# Autodesk Inventor assembly: AluminumProfileMount
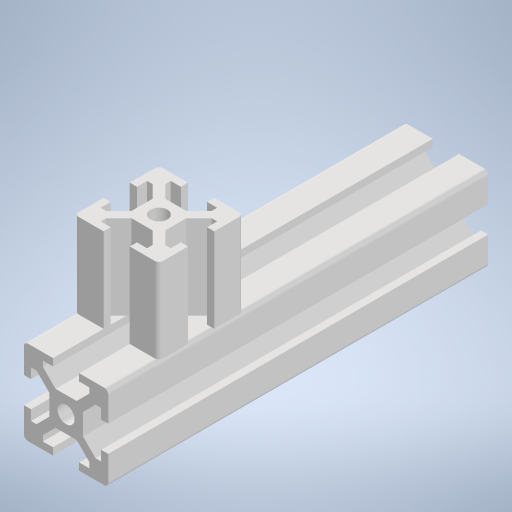
[picture p0: Inventor's stored thumbnail of the model, 512x512]
Saved by Autodesk Inventor 2023 (Build 270158000, 158)
## iProperties
Created: 2024-02-04
Part Number: AluminumProfileMount
Document SubType Name: Assembly
Designer: victo
Author: victo
## Documents named in this file (3)
- C:\Users\victo\Documents\ball-balancing-digital-twin\Mechanics\CAD\AluminumProfileMount.iam
- C:\Users\victo\Documents\ball-balancing-digital-twin\Mechanics\CAD\Aluminum_Profile_202090.ipt
- C:\Users\victo\Documents\ball-balancing-digital-twin\Mechanics\CAD\Aluminum_Profile_202020.ipt
## Components (2 placed, 2 different names)
1. Aluminum_Profile_202090:1 — Mate:1, Flush:1, Flush:2
2. Aluminum_Profile_202020:1 — Mate:1, Flush:1, Flush:2
## Relationships (3: Flush 2, Mate 1)
- Mate:1: Aluminum_Profile_202090:1 ↔ Aluminum_Profile_202020:1
- Flush:1: Aluminum_Profile_202090:1 ↔ Aluminum_Profile_202020:1
- Flush:2 (12 mm): Aluminum_Profile_202090:1 ↔ Aluminum_Profile_202020:1
